# Autodesk Inventor assembly: КВ33-AN1-01-00-Колесо
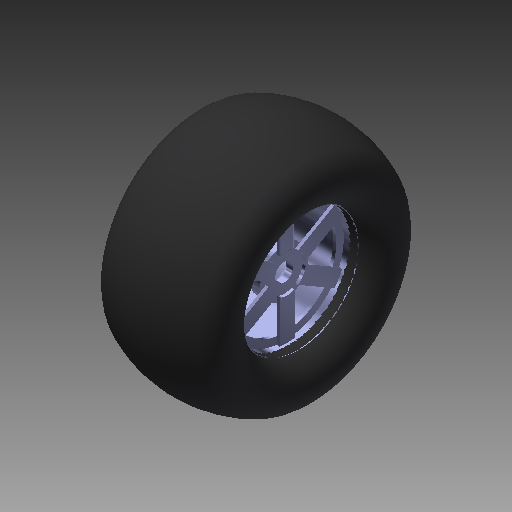
[picture p0: Inventor's stored thumbnail of the model, 512x512]
Saved by Autodesk Inventor 2018 (Build 220112000, 112)
## iProperties
Part Number: КВ33-AN1-01-00-Колесо
Material: Типовые
Document SubType Name: Assembly
Designer: sbnnl
Author: sbnnl
## Documents named in this file (3)
- D:\Загрузки\IMMO\01-00-Колесо.iam
- D:\Загрузки\IMMO\01-02-Диск.ipt
- D:\Загрузки\IMMO\01-01-Шина.ipt
## Components (2 placed, 2 different names)
1. 01-01-Шина:1 — Совмещение:1
2. 01-02-Диск:1 — Совмещение:1
## Relationships (1: Mate 1)
- Совмещение:1 [Mate]: 01-01-Шина:1 ↔ 01-02-Диск:1
